# Autodesk Inventor assembly: Euph Cart
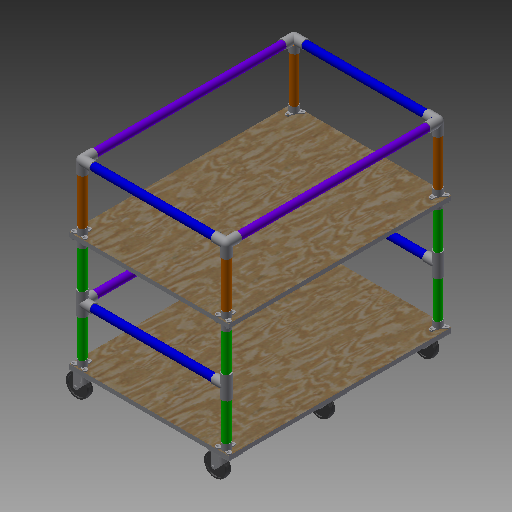
[picture p0: Inventor's stored thumbnail of the model, 512x512]
Saved by Autodesk Inventor 2018.2 (Build 222227000, 227)
## iProperties
Created: 2018-02-07
Part Number: Euph Cart
Document SubType Name: Assembly
Designer: owner
Author: owner
## Documents named in this file (11)
- Z:\The Pickle - 4 - Copy\Final Carts\Euph Cart\Euph Cart.iam
- Z:\The Pickle - 4 - Copy\Final Carts\Stuff Used By All Carts\PVC Fittings (Formufit)\4-way Tee 1 Inch.ipt
- Z:\The Pickle - 4 - Copy\Final Carts\Stuff Used By All Carts\PVC Fittings (Formufit)\Tee 1 Inch.ipt
- Z:\The Pickle - 4 - Copy\Final Carts\Stuff Used By All Carts\PVC Fittings (Formufit)\Wood Mount 1 Inch.ipt
- Z:\The Pickle - 4 - Copy\Final Carts\Euph Cart\Pipe 1.ipt
- Z:\The Pickle - 4 - Copy\Final Carts\Euph Cart\Pipe 2.ipt
- Z:\The Pickle - 4 - Copy\Final Carts\Euph Cart\Pipe 3.ipt
- Z:\The Pickle - 4 - Copy\Final Carts\Euph Cart\Plywood Base - Euph.ipt
- Z:\The Pickle - 4 - Copy\Final Carts\Stuff Used By All Carts\WHEELS.ipt
- Z:\The Pickle - 4 - Copy\Final Carts\Stuff Used By All Carts\PVC Fittings (Formufit)\3-way 90 1 Inch.ipt
- Z:\The Pickle - 4 - Copy\Final Carts\Euph Cart\Pipe 5.ipt
## Components (47 placed, 10 different names)
1. Plywood Base - Euph:2 — Mate:1, Tangent:1, Tangent:2, Tangent:3, Flush:1, Flush:2, Flush:15, Flush:16, Flush:17, Flush:18, Mate:5
2. Plywood Base - Euph:3 — Mate:2, Flush:1, Flush:2, Mate:3, Tangent:4, Tangent:5, Tangent:6
3. WHEELS:1 — Flush:3, Flush:7, Flush:8, Flush:11
4. WHEELS:2 — Flush:4, Flush:6, Flush:7, Flush:9, Flush:11, Flush:12
5. WHEELS:3 — Flush:5, Flush:6, Flush:10, Flush:12, Flush:18
6. WHEELS:4 — Flush:5, Flush:10, Flush:14, Flush:16, Flush:17, Mate:4
7. WHEELS:5 — Flush:4, Flush:9, Flush:13, Flush:14, Mate:4
8. WHEELS:6 — Flush:3, Flush:8, Flush:13, Flush:15, Mate:5
9. Pipe 1:1 — Insert:14, Insert:15
10. Pipe 1:2 — Insert:34, Insert:35
11. Pipe 1:3 — Insert:28, Insert:29
12. Pipe 1:4 — Insert:20, Insert:21
13. Pipe 2:1 — Insert:17, Insert:18
14. Pipe 2:2 — Insert:31, Insert:32
15. Pipe 2:3 — Insert:37
16. Pipe 3:1 — Insert:1, Insert:13
17. Pipe 3:2 — Insert:6, Insert:24
18. Pipe 3:3 — Insert:4, Insert:22
19. Pipe 3:4 — Insert:7, Insert:25
20. Pipe 3:5 — Insert:3, Insert:19
21. Pipe 3:6 — Insert:8, Insert:26
22. Pipe 3:7 — Insert:2, Insert:16
23. Pipe 3:8 — Insert:5, Insert:23
24. Wood Mount 1 Inch:1 — Insert:2
25. Wood Mount 1 Inch:2 — Mate:1, Tangent:1, Tangent:2, Tangent:3, Insert:1
26. Wood Mount 1 Inch:5 — Insert:9, Mate:3, Tangent:4, Tangent:5, Tangent:6
27. Wood Mount 1 Inch:8 — Insert:12
28. Wood Mount 1 Inch:9 — Insert:5, Mate:2
29. Wood Mount 1 Inch:10 — Insert:6
30. 3-way 90 1 Inch:1 — Insert:32, Insert:33, Insert:34
31. 3-way 90 1 Inch:2 — Insert:35, Insert:36, Insert:37
32. 3-way 90 1 Inch:3 — Insert:27, Insert:28
33. 3-way 90 1 Inch:4 — Insert:29, Insert:30, Insert:31
34. 4-way Tee 1 Inch:1 — Insert:18, Insert:19, Insert:20, Insert:25
35. 4-way Tee 1 Inch:2 — Insert:15, Insert:16, Insert:17, Insert:24
36. Tee 1 Inch:1 — Insert:13, Insert:14, Insert:23
37. Tee 1 Inch:2 — Insert:21, Insert:22, Insert:26
38. Wood Mount 1 Inch:13 — Insert:3
39. Wood Mount 1 Inch:14 — Insert:4
40. Wood Mount 1 Inch:15 — Insert:10
41. Wood Mount 1 Inch:16 — Insert:11
42. Wood Mount 1 Inch:17 — Insert:7
43. Wood Mount 1 Inch:18 — Insert:8
44. Pipe 5:1 — Insert:12, Insert:30
45. Pipe 5:2 — Insert:11, Insert:36
46. Pipe 5:3 — Insert:10, Insert:33
47. Pipe 5:4 — Insert:9, Insert:27
## Relationships (66: Insert 37, Flush 18, Tangent 6, Mate 5)
- Mate:1: Plywood Base - Euph:2 ↔ Wood Mount 1 Inch:2
- Tangent:1: Plywood Base - Euph:2 ↔ Wood Mount 1 Inch:2
- Tangent:2: Plywood Base - Euph:2 ↔ Wood Mount 1 Inch:2
- Tangent:3: Plywood Base - Euph:2 ↔ Wood Mount 1 Inch:2
- Insert:1: Pipe 3:1 ↔ Wood Mount 1 Inch:2
- Insert:2: Pipe 3:7 ↔ Wood Mount 1 Inch:1
- Insert:3: Pipe 3:5 ↔ Wood Mount 1 Inch:13
- Insert:4: Pipe 3:3 ↔ Wood Mount 1 Inch:14
- Insert:5: Pipe 3:8 ↔ Wood Mount 1 Inch:9
- Insert:6: Pipe 3:2 ↔ Wood Mount 1 Inch:10
- Insert:7: Pipe 3:4 ↔ Wood Mount 1 Inch:17
- Insert:8: Pipe 3:6 ↔ Wood Mount 1 Inch:18
- Insert:9: Wood Mount 1 Inch:5 ↔ Pipe 5:4
- Insert:10: Wood Mount 1 Inch:15 ↔ Pipe 5:3
- Insert:11: Wood Mount 1 Inch:16 ↔ Pipe 5:2
- Insert:12: Wood Mount 1 Inch:8 ↔ Pipe 5:1
- Insert:13: Pipe 3:1 ↔ Tee 1 Inch:1
- Insert:14: Pipe 1:1 ↔ Tee 1 Inch:1
- Insert:15: Pipe 1:1 ↔ 4-way Tee 1 Inch:2
- Insert:16: Pipe 3:7 ↔ 4-way Tee 1 Inch:2
- Insert:17: Pipe 2:1 ↔ 4-way Tee 1 Inch:2
- Insert:18: Pipe 2:1 ↔ 4-way Tee 1 Inch:1
- Insert:19: Pipe 3:5 ↔ 4-way Tee 1 Inch:1
- Insert:20: Pipe 1:4 ↔ 4-way Tee 1 Inch:1
- Insert:21: Pipe 1:4 ↔ Tee 1 Inch:2
- Insert:22: Pipe 3:3 ↔ Tee 1 Inch:2
- Insert:23: Pipe 3:8 ↔ Tee 1 Inch:1
- Insert:24: Pipe 3:2 ↔ 4-way Tee 1 Inch:2
- Insert:25: Pipe 3:4 ↔ 4-way Tee 1 Inch:1
- Insert:26: Pipe 3:6 ↔ Tee 1 Inch:2
- Mate:2: Plywood Base - Euph:3 ↔ Wood Mount 1 Inch:9
- Flush:1: Plywood Base - Euph:2 ↔ Plywood Base - Euph:3
- Flush:2: Plywood Base - Euph:2 ↔ Plywood Base - Euph:3
- Mate:3: Plywood Base - Euph:3 ↔ Wood Mount 1 Inch:5
- Tangent:4: Plywood Base - Euph:3 ↔ Wood Mount 1 Inch:5
- Tangent:5: Plywood Base - Euph:3 ↔ Wood Mount 1 Inch:5
- Tangent:6: Plywood Base - Euph:3 ↔ Wood Mount 1 Inch:5
- Insert:27: 3-way 90 1 Inch:3 ↔ Pipe 5:4
- Insert:28: Pipe 1:3 ↔ 3-way 90 1 Inch:3
- Insert:29: Pipe 1:3 ↔ 3-way 90 1 Inch:4
- Insert:30: 3-way 90 1 Inch:4 ↔ Pipe 5:1
- Insert:31: Pipe 2:2 ↔ 3-way 90 1 Inch:4
- Insert:32: Pipe 2:2 ↔ 3-way 90 1 Inch:1
- Insert:33: 3-way 90 1 Inch:1 ↔ Pipe 5:3
- Insert:34: Pipe 1:2 ↔ 3-way 90 1 Inch:1
- Insert:35: Pipe 1:2 ↔ 3-way 90 1 Inch:2
- Insert:36: 3-way 90 1 Inch:2 ↔ Pipe 5:2
- Insert:37: Pipe 2:3 ↔ 3-way 90 1 Inch:2
- Flush:3: WHEELS:1 ↔ WHEELS:6
- Flush:4: WHEELS:2 ↔ WHEELS:5
- Flush:5: WHEELS:3 ↔ WHEELS:4
- Flush:6: WHEELS:2 ↔ WHEELS:3
- Flush:7: WHEELS:1 ↔ WHEELS:2
- Flush:8: WHEELS:1 ↔ WHEELS:6
- Flush:9: WHEELS:2 ↔ WHEELS:5
- Flush:10: WHEELS:3 ↔ WHEELS:4
- Flush:11: WHEELS:1 ↔ WHEELS:2
- Flush:12: WHEELS:2 ↔ WHEELS:3
- Flush:13: WHEELS:5 ↔ WHEELS:6
- Flush:14: WHEELS:4 ↔ WHEELS:5
- Flush:15: Plywood Base - Euph:2 ↔ WHEELS:6
- Flush:16: Plywood Base - Euph:2 ↔ WHEELS:4
- Flush:17: Plywood Base - Euph:2 ↔ WHEELS:4
- Flush:18: Plywood Base - Euph:2 ↔ WHEELS:3
- Mate:4 (405.1046 mm): WHEELS:4 ↔ WHEELS:5
- Mate:5: Plywood Base - Euph:2 ↔ WHEELS:6
